# Autodesk Inventor assembly: Basement_And_Basement_And_First_Floor_Transition
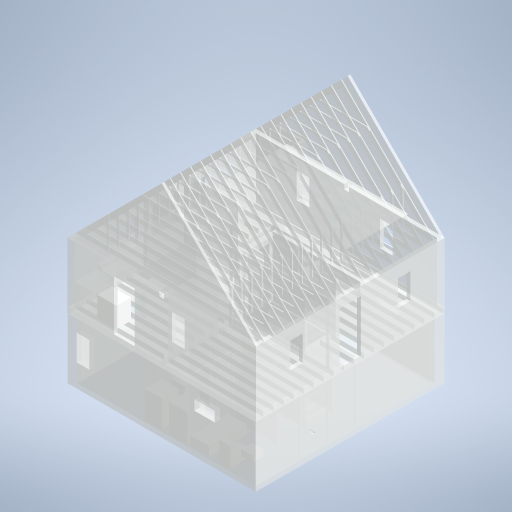
[picture p0: Inventor's stored thumbnail of the model, 512x512]
Saved by Autodesk Inventor 2024 (Build 280153020, 153B)
## iProperties
Created: 2023-05-18
Part Number: Basement_And_Basement_And_First_Floor_Transition
Document SubType Name: Assembly
Designer: Tom
Author: Tom
## Documents named in this file (9)
- C:\Users\Tom\Documents\Tom_Levers_Public_Git_Repository\Inventor\Mobility\Finished_House.iam
- C:\Users\Tom\Documents\Tom_Levers_Public_Git_Repository\Inventor\Mobility\Basement\Finished_Basement.iam
- C:\Users\Tom\Documents\Tom_Levers_Public_Git_Repository\Inventor\Mobility\Transition_For_Finished_Basement_And_First_Floor.ipt
- C:\Users\Tom\Documents\Tom_Levers_Public_Git_Repository\Inventor\Mobility\First_Floor\Finished_First_Floor.iam
- C:\Users\Tom\Documents\Tom_Levers_Public_Git_Repository\Inventor\Mobility\First_Floor\Window_Cabinet\Window_Cabinet.iam
- C:\Users\Tom\Documents\Tom_Levers_Public_Git_Repository\Inventor\Mobility\First_Floor\Range.ipt
- C:\Users\Tom\Documents\Tom_Levers_Public_Git_Repository\Inventor\Mobility\First_Floor\Stairs_Between_First_Floor_And_Second_Floor.ipt
- C:\Users\Tom\Documents\Tom_Levers_Public_Git_Repository\Inventor\Mobility\First_Floor\Beam--7.5_x_7.5_x_300.ipt
- C:\Users\Tom\Documents\Tom_Levers_Public_Git_Repository\Inventor\Mobility\Attic\Finished_Attic.iam
## Components (8 placed, 8 different names)
1. Finished_Basement:1 [sub-assembly] — Mate:1, Flush:1, Flush:2, Flush:3, Flush:4
2. Transition_For_Finished_Basement_And_First_Floor:1 — Mate:1, Flush:1, Flush:2, Mate:5, Mate:7, Mate:10, Mate:11
3. Finished_First_Floor:1 [sub-assembly] — Mate:8, Mate:9, Flush:3, Mate:11, Flush:4, Mate:12, Flush:5, Mate:13, Mate:14, Flush:6, Mate:15
4. Window_Cabinet:1 [sub-assembly] — Mate:5
5. Range:1 — Mate:7
6. Stairs_Between_First_Floor_And_Second_Floor:1 — Mate:8, Mate:9, Mate:10
7. Beam--7.5_x_7.5_x_300:1 — Mate:12, Flush:5, Mate:13
8. Finished_Attic:1 [sub-assembly] — Mate:14, Flush:6, Mate:15
## Relationships (17: Mate 11, Flush 6)
- Mate:1: Finished_Basement:1 ↔ Transition_For_Finished_Basement_And_First_Floor:1
- Flush:1: Finished_Basement:1 ↔ Transition_For_Finished_Basement_And_First_Floor:1
- Flush:2 (215.9 mm): Finished_Basement:1 ↔ Transition_For_Finished_Basement_And_First_Floor:1
- Mate:5: Transition_For_Finished_Basement_And_First_Floor:1 ↔ Window_Cabinet:1
- Mate:7: Transition_For_Finished_Basement_And_First_Floor:1 ↔ Range:1
- Mate:8 (1244.6 mm): Finished_First_Floor:1 ↔ Stairs_Between_First_Floor_And_Second_Floor:1
- Mate:9: Finished_First_Floor:1 ↔ Stairs_Between_First_Floor_And_Second_Floor:1
- Mate:10: Transition_For_Finished_Basement_And_First_Floor:1 ↔ Stairs_Between_First_Floor_And_Second_Floor:1
- Flush:3: Finished_Basement:1 ↔ Finished_First_Floor:1
- Mate:11: Transition_For_Finished_Basement_And_First_Floor:1 ↔ Finished_First_Floor:1
- Flush:4 (215.9 mm): Finished_Basement:1 ↔ Finished_First_Floor:1
- Mate:12: Finished_First_Floor:1 ↔ Beam--7.5_x_7.5_x_300:1
- Flush:5: Finished_First_Floor:1 ↔ Beam--7.5_x_7.5_x_300:1
- Mate:13: Finished_First_Floor:1 ↔ Beam--7.5_x_7.5_x_300:1
- Mate:14: Finished_First_Floor:1 ↔ Finished_Attic:1
- Flush:6: Finished_First_Floor:1 ↔ Finished_Attic:1
- Mate:15 (-3810 mm): Finished_First_Floor:1 ↔ Finished_Attic:1
## Named parameters: sa_0 = 980.999, sa_1 = 19.1674, sa_2 = 19.1674
note: some values were not read from the file. Shown as the stored number, unit unknown: "sa_0", "sa_1", "sa_2".
